# Autodesk Inventor assembly: headstage+flex connector_MIR
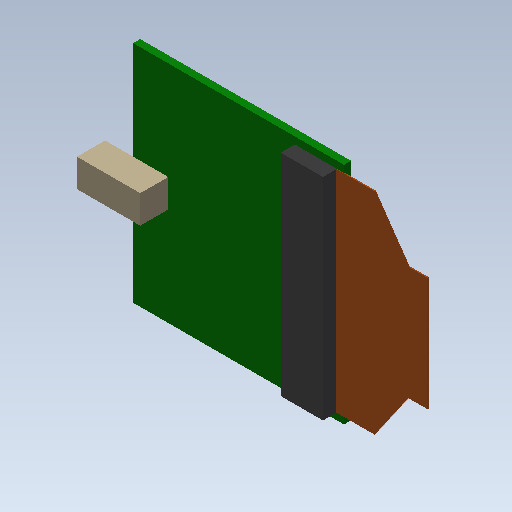
[picture p0: Inventor's stored thumbnail of the model, 512x512]
Saved by Autodesk Inventor 2020 (Build 240168000, 168)
## iProperties
Created: 2020-03-27
Part Number: headstage+flex connector_MIR
Document SubType Name: Assembly
Designer: Thomas Zhihao Luo
Author: Thomas Zhihao Luo
## Documents named in this file (3)
- C:\Users\Thomas Zhihao Luo\Desktop\NEW\headstage+flex connector_MIR.iam
- C:\Users\Thomas Zhihao Luo\Desktop\NEW\headstage_MIR.ipt
- C:\Users\Thomas Zhihao Luo\Desktop\NEW\flexcable3_MIR.ipt
## Components (2 placed, 2 different names)
1. headstage_MIR:1 — Rigid:1
2. flexcable3_MIR:1 — Rigid:1
## Relationships (1: WeldJoint 1)
- Rigid:1 [WeldJoint]: headstage_MIR:1 ↔ flexcable3_MIR:1
